# Autodesk Inventor assembly: chassis
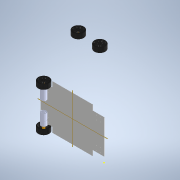
[picture p0: Inventor's stored thumbnail of the model, 180x180]
Saved by Autodesk Inventor 2022 (Build 260153000, 153)
## iProperties
Created: 2023-03-16
Part Number: chassis
Document SubType Name: Assembly
Designer: JOU
Author: JOU
## Documents named in this file (6)
- C:\Users\JOU\Desktop\git\Areo_Rider_Cabin\car\chassis.iam
- C:\Users\JOU\Desktop\git\Areo_Rider_Cabin\car\base.ipt
- C:\Users\JOU\Desktop\git\Areo_Rider_Cabin\car\motor_base.ipt
- C:\Users\JOU\Desktop\git\Areo_Rider_Cabin\motor\25GA370.ipt
- C:\Users\JOU\Desktop\git\Areo_Rider_Cabin\car\Coupling.ipt
- C:\Users\JOU\Desktop\git\Areo_Rider_Cabin\car\wheel.ipt
## Components (13 placed, 5 different names)
1. base:1 — 貼合:1, 貼合:2, 貼合:5, 貼合:6, 貼合:7, 貼合:8
2. motor_base:1 — 貼合:1, 貼合:5, 貼合:6, 貼合:16, 貼合:17, 貼合:18
3. motor_base:2 — 貼合:2, 貼合:7, 貼合:8, 貼合:13, 貼合:14, 貼合:15
4. 25GA370:1 — 貼合:13, 貼合:14, 貼合:15, 貼合:33, 貼合:34
5. 25GA370:3 — 貼合:16, 貼合:17, 貼合:18, 貼合:22, 貼合:23
6. Coupling:1 — 貼合:19, 貼合:20, 貼合:21, 貼合:22, 貼合:23
7. wheel:1 — 貼合:19, 貼合:20, 貼合:21
8. Coupling:2
9. wheel:2
10. Coupling:3
11. wheel:3
12. Coupling:4 — 貼合:33, 貼合:34
13. wheel:4
## Relationships (28: Mate 28)
- 貼合:1 [Mate]: base:1 ↔ motor_base:1
- 貼合:2 [Mate]: base:1 ↔ motor_base:2
- 貼合:5 [Mate]: base:1 ↔ motor_base:1
- 貼合:6 [Mate]: base:1 ↔ motor_base:1
- 貼合:7 [Mate]: base:1 ↔ motor_base:2
- 貼合:8 [Mate]: base:1 ↔ motor_base:2
- 貼合:13 [Mate]: motor_base:2 ↔ 25GA370:1
- 貼合:14 [Mate]: motor_base:2 ↔ 25GA370:1
- 貼合:15 [Mate]: motor_base:2 ↔ 25GA370:1
- 貼合:16 [Mate]: motor_base:1 ↔ 25GA370:3
- 貼合:17 [Mate]: motor_base:1 ↔ 25GA370:3
- 貼合:18 [Mate]: motor_base:1 ↔ 25GA370:3
- 貼合:19 [Mate]: Coupling:1 ↔ wheel:1
- 貼合:20 [Mate]: Coupling:1 ↔ wheel:1
- 貼合:21 [Mate]: Coupling:1 ↔ wheel:1
- 貼合:22 [Mate]: 25GA370:3 ↔ Coupling:1
- 貼合:23 [Mate]: 25GA370:3 ↔ Coupling:1
- [Mate]: Coupling:2 ↔ wheel:2
- [Mate]: Coupling:2 ↔ wheel:2
- [Mate]: Coupling:2 ↔ wheel:2
- [Mate]: Coupling:3 ↔ wheel:3
- [Mate]: Coupling:3 ↔ wheel:3
- [Mate]: Coupling:3 ↔ wheel:3
- [Mate]: Coupling:4 ↔ wheel:4
- [Mate]: Coupling:4 ↔ wheel:4
- [Mate]: Coupling:4 ↔ wheel:4
- 貼合:33 [Mate]: 25GA370:1 ↔ Coupling:4
- 貼合:34 [Mate]: 25GA370:1 ↔ Coupling:4
## Named parameters: d26_d21 = 0 mm, d27_d22 = 0 mm, d28_d23 = 0 mm, d29_d21 = 0 mm, d30_d22 = 0 mm, d31_d23 = 0 mm, d32_d21 = 0 mm, d33_d22 = 0 mm, d34_d23 = 0 mm
